# Autodesk Inventor assembly: Weight Assembly
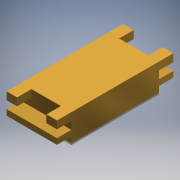
[picture p0: Inventor's stored thumbnail of the model, 180x180]
Saved by Autodesk Inventor 2019.4 (Build 234330000, 330)
## iProperties
Created: 2021-03-04
Part Number: Weight Assembly
Document SubType Name: Assembly
Designer: caleb
Author: caleb
## Documents named in this file (3)
- C:\Users\cfang\Desktop\nebraska-silicon-lab\Hardware\ETL\Module Assembly\Weight\Weight Assembly.iam
- C:\Users\cfang\Desktop\nebraska-silicon-lab\Hardware\ETL\Module Assembly\Weight\Weight Body.ipt
- C:\Users\cfang\Desktop\nebraska-silicon-lab\Hardware\ETL\Module Assembly\Weight\Bottom Surface.ipt
## Components (2 placed, 2 different names)
1. Weight Body:1 — Insert:1, Mate:1
2. Bottom Surface:1 — Insert:1, Mate:1
## Relationships (2: Insert 1, Mate 1)
- Insert:1: Weight Body:1 ↔ Bottom Surface:1
- Mate:1: Weight Body:1 ↔ Bottom Surface:1
